# Autodesk Inventor assembly: Tesla_Coul
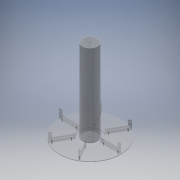
[picture p0: Inventor's stored thumbnail of the model, 180x180]
Saved by Autodesk Inventor 2016 (Build 200138000, 138)
## iProperties
Created: 2018-04-27
Part Number: Tesla_Coul
Document SubType Name: Assembly
Designer: Phil Erle
Author: Phil Erle
## Documents named in this file (8)
- C:\Users\Phil Erle\Desktop\Adrastea\Tesla_Coul.iam
- C:\Users\Phil Erle\Desktop\Adrastea\primary_holder.ipt
- C:\Users\Phil Erle\Desktop\Adrastea\Secondary.ipt
- C:\Users\Phil Erle\Desktop\Adrastea\Seconday_End_Bottom.ipt
- C:\Users\Phil Erle\Desktop\Adrastea\Seconday_End_Top.ipt
- C:\Users\Phil Erle\Desktop\Adrastea\Primary.ipt
- C:\Users\Phil Erle\Desktop\Adrastea\Normteile\Muttern\mutter_din934_m4-10.ipt
- C:\Users\Phil Erle\Desktop\Adrastea\Normteile\Schrauben\M4\Zylinderkopf\din_en_iso_4762_m4x16.ipt
## Components (34 placed, 7 different names)
1. primary_holder:1 — Mate:9, Mate:57, Mate:59, Flush:4, Angle:1, Mate:76, Mate:77
2. primary_holder:2 — Mate:8, Mate:48, Mate:49, Mate:50, Mate:51, Flush:6
3. primary_holder:3 — Mate:7, Mate:58, Mate:62, Mate:63, Mate:66, Flush:5
4. primary_holder:4 — Mate:6, Mate:56, Mate:60, Mate:64, Mate:65, Mate:69
5. primary_holder:5 — Mate:5, Mate:55, Mate:61, Flush:3, Mate:74, Mate:75
6. primary_holder:6 — Mate:4, Mate:52, Mate:53, Mate:70, Mate:72, Mate:73
7. Secondary:1 — Mate:3, Mate:11, Mate:12, Mate:13, Mate:79
8. Seconday_End_Bottom:1 — Mate:1, Mate:2, Flush:1, Mate:3, Mate:10, Mate:11, Flush:2
9. Seconday_End_Top:1 — Mate:12, Mate:13, Mate:78
10. Primary:1 — Mate:4, Mate:5, Mate:6, Mate:7, Mate:8, Mate:9, Mate:10, Flush:2, Mate:14, Mate:15, Mate:16, Mate:17, Mate:18, Mate:19, Mate:20, Mate:21, Mate:22, Mate:23, Mate:24, Mate:25, Mate:38, Mate:39, Mate:40, Mate:41, Mate:42, Mate:43, Mate:44, Mate:45, Mate:46, Mate:47, Mate:54, Mate:71
11. mutter_din934_m4-10:1 — Mate:27, Mate:57, Mate:77
12. mutter_din934_m4-10:2 — Mate:28, Mate:62, Mate:63
13. mutter_din934_m4-10:3 — Mate:26, Mate:59, Mate:76
14. mutter_din934_m4-10:4 — Mate:36, Mate:52, Mate:72
15. mutter_din934_m4-10:5 — Mate:30, Mate:48, Mate:50
16. mutter_din934_m4-10:6 — Mate:37, Mate:53, Mate:73
17. mutter_din934_m4-10:7 — Mate:33, Mate:61, Mate:75
18. mutter_din934_m4-10:8 — Mate:34, Mate:55, Mate:74
19. mutter_din934_m4-10:9 — Mate:32, Mate:56, Mate:64
20. mutter_din934_m4-10:10 — Mate:31, Mate:60, Mate:65
21. mutter_din934_m4-10:11 — Mate:35, Mate:49, Mate:51
22. mutter_din934_m4-10:12 — Mate:29, Mate:58, Mate:66
23. din_en_iso_4762_m4x16:1 — Mate:14, Mate:27, Mate:42
24. din_en_iso_4762_m4x16:2 — Mate:15, Mate:26, Mate:39
25. din_en_iso_4762_m4x16:3 — Mate:16, Mate:36, Mate:40
26. din_en_iso_4762_m4x16:4 — Mate:17, Mate:37, Mate:46
27. din_en_iso_4762_m4x16:5 — Mate:24, Mate:35, Mate:45
28. din_en_iso_4762_m4x16:6 — Mate:25, Mate:30, Mate:44
29. din_en_iso_4762_m4x16:7 — Mate:23, Mate:34
30. din_en_iso_4762_m4x16:8 — Mate:22, Mate:33, Mate:47
31. din_en_iso_4762_m4x16:9 — Mate:21, Mate:32, Mate:71
32. din_en_iso_4762_m4x16:10 — Mate:20, Mate:31, Mate:43
33. din_en_iso_4762_m4x16:11 — Mate:18, Mate:29, Mate:38
34. din_en_iso_4762_m4x16:12 — Mate:19, Mate:28, Mate:41
## Relationships (87: Mate 79, Flush 6, Angle 2)
- Mate:1: Seconday_End_Bottom:1
- Mate:2: Seconday_End_Bottom:1
- Flush:1: Seconday_End_Bottom:1
- Mate:3: Secondary:1 ↔ Seconday_End_Bottom:1
- Mate:4: primary_holder:6 ↔ Primary:1
- Mate:5: primary_holder:5 ↔ Primary:1
- Mate:6: primary_holder:4 ↔ Primary:1
- Mate:7: primary_holder:3 ↔ Primary:1
- Mate:8: primary_holder:2 ↔ Primary:1
- Mate:9: primary_holder:1 ↔ Primary:1
- Mate:10: Seconday_End_Bottom:1 ↔ Primary:1
- Mate:11: Secondary:1 ↔ Seconday_End_Bottom:1
- Mate:12: Secondary:1 ↔ Seconday_End_Top:1
- Mate:13: Secondary:1 ↔ Seconday_End_Top:1
- Flush:2: Seconday_End_Bottom:1 ↔ Primary:1
- Mate:14: Primary:1 ↔ din_en_iso_4762_m4x16:1
- Mate:15: Primary:1 ↔ din_en_iso_4762_m4x16:2
- Mate:16: Primary:1 ↔ din_en_iso_4762_m4x16:3
- Mate:17: Primary:1 ↔ din_en_iso_4762_m4x16:4
- Mate:18: Primary:1 ↔ din_en_iso_4762_m4x16:11
- Mate:19: Primary:1 ↔ din_en_iso_4762_m4x16:12
- Mate:20: Primary:1 ↔ din_en_iso_4762_m4x16:10
- Mate:21: Primary:1 ↔ din_en_iso_4762_m4x16:9
- Mate:22: Primary:1 ↔ din_en_iso_4762_m4x16:8
- Mate:23: Primary:1 ↔ din_en_iso_4762_m4x16:7
- Mate:24: Primary:1 ↔ din_en_iso_4762_m4x16:5
- Mate:25: Primary:1 ↔ din_en_iso_4762_m4x16:6
- Mate:26: mutter_din934_m4-10:3 ↔ din_en_iso_4762_m4x16:2
- Mate:27: mutter_din934_m4-10:1 ↔ din_en_iso_4762_m4x16:1
- Mate:28: mutter_din934_m4-10:2 ↔ din_en_iso_4762_m4x16:12
- Mate:29: mutter_din934_m4-10:12 ↔ din_en_iso_4762_m4x16:11
- Mate:30: mutter_din934_m4-10:5 ↔ din_en_iso_4762_m4x16:6
- Mate:31: mutter_din934_m4-10:10 ↔ din_en_iso_4762_m4x16:10
- Mate:32: mutter_din934_m4-10:9 ↔ din_en_iso_4762_m4x16:9
- Mate:33: mutter_din934_m4-10:7 ↔ din_en_iso_4762_m4x16:8
- Mate:34: mutter_din934_m4-10:8 ↔ din_en_iso_4762_m4x16:7
- Mate:35: mutter_din934_m4-10:11 ↔ din_en_iso_4762_m4x16:5
- Mate:36: mutter_din934_m4-10:4 ↔ din_en_iso_4762_m4x16:3
- Mate:37: mutter_din934_m4-10:6 ↔ din_en_iso_4762_m4x16:4
- Mate:38: Primary:1 ↔ din_en_iso_4762_m4x16:11
- Mate:39: Primary:1 ↔ din_en_iso_4762_m4x16:2
- Mate:40: Primary:1 ↔ din_en_iso_4762_m4x16:3
- Mate:41: Primary:1 ↔ din_en_iso_4762_m4x16:12
- Mate:42: Primary:1 ↔ din_en_iso_4762_m4x16:1
- Mate:43: Primary:1 ↔ din_en_iso_4762_m4x16:10
- Mate:44: Primary:1 ↔ din_en_iso_4762_m4x16:6
- Mate:45: Primary:1 ↔ din_en_iso_4762_m4x16:5
- Mate:46: Primary:1 ↔ din_en_iso_4762_m4x16:4
- Mate:47: Primary:1 ↔ din_en_iso_4762_m4x16:8
- Mate:48: primary_holder:2 ↔ mutter_din934_m4-10:5
- Mate:49: primary_holder:2 ↔ mutter_din934_m4-10:11
- Mate:50: primary_holder:2 ↔ mutter_din934_m4-10:5
- Mate:51: primary_holder:2 ↔ mutter_din934_m4-10:11
- Mate:52: primary_holder:6 ↔ mutter_din934_m4-10:4
- Mate:53: primary_holder:6 ↔ mutter_din934_m4-10:6
- Mate:54: Primary:1
- Mate:55: primary_holder:5 ↔ mutter_din934_m4-10:8
- Mate:56: primary_holder:4 ↔ mutter_din934_m4-10:9
- Mate:57: primary_holder:1 ↔ mutter_din934_m4-10:1
- Mate:58: primary_holder:3 ↔ mutter_din934_m4-10:12
- Mate:59: primary_holder:1 ↔ mutter_din934_m4-10:3
- Mate:60: primary_holder:4 ↔ mutter_din934_m4-10:10
- Mate:61: primary_holder:5 ↔ mutter_din934_m4-10:7
- Mate:62: primary_holder:3 ↔ mutter_din934_m4-10:2
- Mate:63: primary_holder:3 ↔ mutter_din934_m4-10:2
- Mate:64: primary_holder:4 ↔ mutter_din934_m4-10:9
- Mate:65: primary_holder:4 ↔ mutter_din934_m4-10:10
- Mate:66: primary_holder:3 ↔ mutter_din934_m4-10:12
- Flush:3 (2.5 mm): primary_holder:5
- Flush:4 (2.5 mm): primary_holder:1
- Mate:67
- Angle:1 (60 deg): primary_holder:1
- Flush:5 (2.5 mm): primary_holder:3
- Flush:6 (2.5 mm): primary_holder:2
- Mate:68
- Angle:2 (-60 deg)
- Mate:69 (-2.5 mm): primary_holder:4
- Mate:70 (-2.5 mm): primary_holder:6
- Mate:71: Primary:1 ↔ din_en_iso_4762_m4x16:9
- Mate:72: primary_holder:6 ↔ mutter_din934_m4-10:4
- Mate:73: primary_holder:6 ↔ mutter_din934_m4-10:6
- Mate:74: primary_holder:5 ↔ mutter_din934_m4-10:8
- Mate:75: primary_holder:5 ↔ mutter_din934_m4-10:7
- Mate:76: primary_holder:1 ↔ mutter_din934_m4-10:3
- Mate:77: primary_holder:1 ↔ mutter_din934_m4-10:1
- Mate:78: Seconday_End_Top:1
- Mate:79: Secondary:1
